# Autodesk Inventor assembly: Battery Pack - Samsung 25R
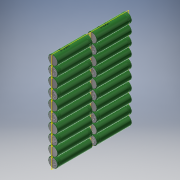
[picture p0: Inventor's stored thumbnail of the model, 180x180]
Saved by Autodesk Inventor 2019.2 (Build 232265000, 265)
## iProperties
Created: 2019-03-02
Part Number: Battery Pack - Samsung 25R
Document SubType Name: Assembly
Designer: Petar
Author: Petar
## Documents named in this file (2)
- D:\OMG\E-Board\CAD\Inventor\Electrical Components\Battery Pack - Samsung 25R.iam
- D:\OMG\E-Board\CAD\Inventor\Electrical Components\Battery Cell - Samsung.ipt
## Components (20 placed, 1 different names)
1. Battery Cell - Samsung:1 — Tangent:1, Flush:1, Flush:2, Mate:3
2. Battery Cell - Samsung:2 — Tangent:1, Flush:1, Flush:2, Tangent:3, Flush:5, Flush:6
3. Battery Cell - Samsung:3 — Tangent:3, Flush:5, Flush:6
4. Battery Cell - Samsung:4 — Tangent:7, Flush:13, Flush:14
5. Battery Cell - Samsung:5 — Tangent:7, Flush:13, Flush:14
6. Battery Cell - Samsung:6
7. Battery Cell - Samsung:7
8. Battery Cell - Samsung:8 — Tangent:9, Flush:17, Flush:18
9. Battery Cell - Samsung:9 — Tangent:9, Flush:17, Flush:18
10. Battery Cell - Samsung:10 — Mate:1, Mate:2
11. Battery Cell - Samsung:11 — Mate:3
12. Battery Cell - Samsung:12
13. Battery Cell - Samsung:13
14. Battery Cell - Samsung:14
15. Battery Cell - Samsung:15
16. Battery Cell - Samsung:16
17. Battery Cell - Samsung:17
18. Battery Cell - Samsung:18
19. Battery Cell - Samsung:19
20. Battery Cell - Samsung:20 — Mate:1, Mate:2
## Relationships (57: Flush 36, Tangent 18, Mate 3)
- Tangent:1: Battery Cell - Samsung:1 ↔ Battery Cell - Samsung:2
- Flush:1: Battery Cell - Samsung:1 ↔ Battery Cell - Samsung:2
- Flush:2: Battery Cell - Samsung:1 ↔ Battery Cell - Samsung:2
- [Tangent]: Battery Cell - Samsung:3 ↔ Battery Cell - Samsung:4
- [Flush]: Battery Cell - Samsung:3 ↔ Battery Cell - Samsung:4
- [Flush]: Battery Cell - Samsung:3 ↔ Battery Cell - Samsung:4
- Tangent:3: Battery Cell - Samsung:2 ↔ Battery Cell - Samsung:3
- Flush:5: Battery Cell - Samsung:2 ↔ Battery Cell - Samsung:3
- Flush:6: Battery Cell - Samsung:2 ↔ Battery Cell - Samsung:3
- [Tangent]: Battery Cell - Samsung:5 ↔ Battery Cell - Samsung:6
- [Flush]: Battery Cell - Samsung:5 ↔ Battery Cell - Samsung:6
- [Flush]: Battery Cell - Samsung:5 ↔ Battery Cell - Samsung:6
- [Tangent]: Battery Cell - Samsung:7 ↔ Battery Cell - Samsung:8
- [Flush]: Battery Cell - Samsung:7 ↔ Battery Cell - Samsung:8
- [Flush]: Battery Cell - Samsung:7 ↔ Battery Cell - Samsung:8
- [Tangent]: Battery Cell - Samsung:6 ↔ Battery Cell - Samsung:7
- [Flush]: Battery Cell - Samsung:6 ↔ Battery Cell - Samsung:7
- [Flush]: Battery Cell - Samsung:6 ↔ Battery Cell - Samsung:7
- Tangent:7: Battery Cell - Samsung:4 ↔ Battery Cell - Samsung:5
- Flush:13: Battery Cell - Samsung:4 ↔ Battery Cell - Samsung:5
- Flush:14: Battery Cell - Samsung:4 ↔ Battery Cell - Samsung:5
- [Tangent]: Battery Cell - Samsung:9 ↔ Battery Cell - Samsung:10
- [Flush]: Battery Cell - Samsung:9 ↔ Battery Cell - Samsung:10
- [Flush]: Battery Cell - Samsung:9 ↔ Battery Cell - Samsung:10
- Tangent:9: Battery Cell - Samsung:8 ↔ Battery Cell - Samsung:9
- Flush:17: Battery Cell - Samsung:8 ↔ Battery Cell - Samsung:9
- Flush:18: Battery Cell - Samsung:8 ↔ Battery Cell - Samsung:9
- [Tangent]: Battery Cell - Samsung:11 ↔ Battery Cell - Samsung:12
- [Flush]: Battery Cell - Samsung:11 ↔ Battery Cell - Samsung:12
- [Flush]: Battery Cell - Samsung:11 ↔ Battery Cell - Samsung:12
- [Tangent]: Battery Cell - Samsung:13 ↔ Battery Cell - Samsung:14
- [Flush]: Battery Cell - Samsung:13 ↔ Battery Cell - Samsung:14
- [Flush]: Battery Cell - Samsung:13 ↔ Battery Cell - Samsung:14
- [Tangent]: Battery Cell - Samsung:12 ↔ Battery Cell - Samsung:13
- [Flush]: Battery Cell - Samsung:12 ↔ Battery Cell - Samsung:13
- [Flush]: Battery Cell - Samsung:12 ↔ Battery Cell - Samsung:13
- [Tangent]: Battery Cell - Samsung:15 ↔ Battery Cell - Samsung:16
- [Flush]: Battery Cell - Samsung:15 ↔ Battery Cell - Samsung:16
- [Flush]: Battery Cell - Samsung:15 ↔ Battery Cell - Samsung:16
- [Tangent]: Battery Cell - Samsung:17 ↔ Battery Cell - Samsung:18
- [Flush]: Battery Cell - Samsung:17 ↔ Battery Cell - Samsung:18
- [Flush]: Battery Cell - Samsung:17 ↔ Battery Cell - Samsung:18
- [Tangent]: Battery Cell - Samsung:16 ↔ Battery Cell - Samsung:17
- [Flush]: Battery Cell - Samsung:16 ↔ Battery Cell - Samsung:17
- [Flush]: Battery Cell - Samsung:16 ↔ Battery Cell - Samsung:17
- [Tangent]: Battery Cell - Samsung:14 ↔ Battery Cell - Samsung:15
- [Flush]: Battery Cell - Samsung:14 ↔ Battery Cell - Samsung:15
- [Flush]: Battery Cell - Samsung:14 ↔ Battery Cell - Samsung:15
- [Tangent]: Battery Cell - Samsung:19 ↔ Battery Cell - Samsung:20
- [Flush]: Battery Cell - Samsung:19 ↔ Battery Cell - Samsung:20
- [Flush]: Battery Cell - Samsung:19 ↔ Battery Cell - Samsung:20
- [Tangent]: Battery Cell - Samsung:18 ↔ Battery Cell - Samsung:19
- [Flush]: Battery Cell - Samsung:18 ↔ Battery Cell - Samsung:19
- [Flush]: Battery Cell - Samsung:18 ↔ Battery Cell - Samsung:19
- Mate:1 (8 mm): Battery Cell - Samsung:10 ↔ Battery Cell - Samsung:20
- Mate:2: Battery Cell - Samsung:10 ↔ Battery Cell - Samsung:20
- Mate:3: Battery Cell - Samsung:1 ↔ Battery Cell - Samsung:11
## Named parameters: d4_d1 = 0 mm, d5_d3 = 0 mm, d6_d0 = 0 mm, d10_d1 = 0 mm, d11_d3 = 0 mm, d12_d4_d1 = 0 mm, d13_d5_d3 = 0 mm, d14_d6_d0 = 0 mm, d15_d7 = 0 mm, d16_d8 = 0 mm, d17_d9 = 0 mm, d18_d0 = 0 mm, d22_d12_d4_d1 = 0 mm, d23_d13_d5_d3 = 0 mm, d24_d14_d6_d0 = 0 mm, d28_d1 = 0 mm, d29_d3 = 0 mm, d30_d4_d1 = 0 mm, d31_d5_d3 = 0 mm, d32_d6_d0 = 0 mm, d33_d7 = 0 mm, d34_d8 = 0 mm, d35_d9 = 0 mm, d36_d10_d1 = 0 mm, d37_d11_d3 = 0 mm, d38_d12_d4_d1 = 0 mm, d39_d13_d5_d3 = 0 mm, d40_d14_d6_d0 = 0 mm, d41_d15_d7 = 0 mm, d42_d16_d8 = 0 mm, d43_d17_d9 = 0 mm, d44_d18_d0 = 0 mm, d45_d19 = 0 mm, d46_d20 = 0 mm, d47_d21 = 0 mm, d48_d22_d12_d4_d1 = 0 mm, d49_d23_d13_d5_d3 = 0 mm, d50_d24_d14_d6_d0 = 0 mm, d51_d25 = 0 mm, d52_d26 = 0 mm, d53_d27 = 0 mm, d54_d0 = 0 mm
